# Autodesk Inventor assembly: 200-40-BOGIE-CONNECTOR-REINFORCEMENT-02
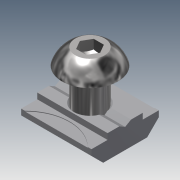
[picture p0: Inventor's stored thumbnail of the model, 180x180]
Saved by Autodesk Inventor 2018.2 (Build 222227000, 227)
## iProperties
Manager: feesmrt
Company: FRANCOR
Part Number: 200-40-BOGIE-CONNECTOR-REINFORCEMENT-02
Project: Rescue Robot
Cost Center: -
Material: Generisch
Document SubType Name: Assembly
Designer: feesmrt
Engineer: feesmrt
Authority: feesmrt
Description: Bogie Connector Reinforcement Screws
Stock Number: 200-40-BOGIE-CONNECTOR-REINFORCEMENT-02
Subject: Rescue Robot
Author: feesmrt
Revision Number: 1
Title: Bogie Connector Reinforcement Screws
## Documents named in this file (3)
- D:\Programmierung\FRANC0R\CAD\02-Rocker-Bogie-Robot\200-ROCKER-BOGIE\200-40-BOGIE-CONNECTOR\200-40-BOGIE-CONNECTOR-REINFORCEMENT-02.iam
- D:\Programmierung\FRANC0R\CAD\02-Rocker-Bogie-Robot\900-COMPONENTS\900-40-SCREWS\900-40-SCREWS-ISO7830_M5x10.ipt
- D:\Programmierung\FRANC0R\CAD\02-Rocker-Bogie-Robot\900-COMPONENTS\900-50-PROFILES\900-50-PROFILES-CONN-N6xM5.ipt
## Components (2 placed, 2 different names)
1. 900-40-SCREWS-ISO7830_M5x10:1 — Passend:1, Passend:2
2. 900-50-PROFILES-CONN-N6xM5:1 — Passend:1, Passend:2, Passend:3
## Relationships (3: Mate 3)
- Passend:1 [Mate]: 900-40-SCREWS-ISO7830_M5x10:1 ↔ 900-50-PROFILES-CONN-N6xM5:1
- Passend:2 [Mate] (6.5 mm): 900-40-SCREWS-ISO7830_M5x10:1 ↔ 900-50-PROFILES-CONN-N6xM5:1
- Passend:3 [Mate]: 900-50-PROFILES-CONN-N6xM5:1
